# Autodesk Inventor assembly: Slides
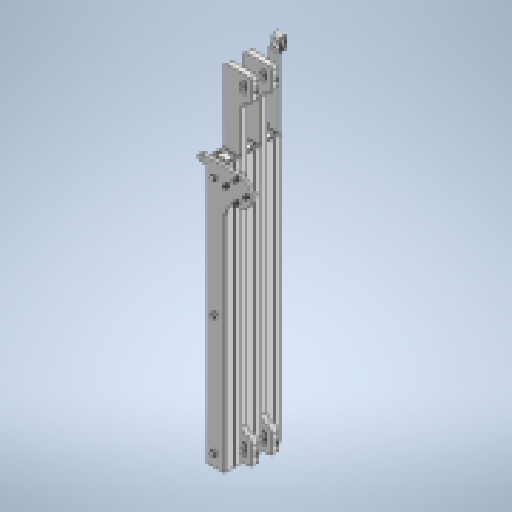
[picture p0: Inventor's stored thumbnail of the model, 512x512]
Saved by Autodesk Inventor 2023 (Build 270158000, 158)
## iProperties
Created: 2022-09-10
Part Number: Slides
Document SubType Name: Assembly
Designer: deli
Author: deli
## Documents named in this file (11)
- C:\Users\deli\OneDrive - Eastside Preparatory School\FTC\8103-power-play\CAD\Slides.iam
- C:\Users\deli\OneDrive - Eastside Preparatory School\FTC\8103-power-play\CAD\FTC-parts\Middle Slide.ipt
- C:\Users\deli\OneDrive - Eastside Preparatory School\FTC\8103-power-play\CAD\FTC-parts\KC-362-30.iam
- C:\Users\deli\OneDrive - Eastside Preparatory School\FTC\8103-power-play\CAD\FTC-parts\LBracket.ipt
- C:\Users\deli\OneDrive - Eastside Preparatory School\FTC\8103-power-play\CAD\ServoMountPlate.ipt
- C:\Users\deli\OneDrive - Eastside Preparatory School\FTC\8103-power-play\CAD\FTC-parts\goBILDA\m3LockNute.ipt
- C:\Users\deli\OneDrive - Eastside Preparatory School\FTC\8103-power-play\CAD\FTC-parts\goBILDA\2800-0004-0008.ipt
- C:\Users\deli\OneDrive - Eastside Preparatory School\FTC\8103-power-play\CAD\FTC-parts\M3\hex_socket_button_head_M3x20.ipt
- C:\Users\deli\OneDrive - Eastside Preparatory School\FTC\8103-power-play\CAD\FTC-parts\LongRobotics\3x12x4mm-bearing.ipt
- C:\Users\deli\OneDrive - Eastside Preparatory School\FTC\8103-power-play\CAD\FTC-parts\goBILDA\2812-0004-0007.ipt
- C:\Users\deli\OneDrive - Eastside Preparatory School\FTC\8103-power-play\CAD\FTC-parts\goBILDA\3408-0001-0001 assembly.ipt
## Components (27 placed, 10 different names)
1. Middle Slide:1
2. KC-362-30:1 [sub-assembly]
3. Middle Slide:2
4. KC-362-30:2 [sub-assembly]
5. KC-362-30:3 [sub-assembly] — Mate:15, Mate:16, Mate:17
6. LBracket:1 — Mate:18, Mate:19, Mate:20, Mate:21, Mate:52, Mate:53, Mate:54, Mate:55, Mate:56, Mate:57, Flush:2
7. ServoMountPlate:1 — Mate:15, Mate:16, Mate:17, Mate:22, Mate:23, Mate:24, Mate:25, Mate:26, Mate:27, Mate:28, Mate:29, Mate:46, Mate:47, Mate:48, Mate:49, Mate:50, Mate:51
8. m3LockNute:1 — Mate:18, Mate:19
9. m3LockNute:2 — Mate:20, Mate:21
10. 2800-0004-0008:1 — Mate:22, Mate:28
11. 2800-0004-0008:2 — Mate:24, Mate:27
12. 2800-0004-0008:3 — Mate:23, Mate:29
13. 2800-0004-0008:4 — Mate:25, Mate:26
14. hex_socket_button_head_M3x20:1
15. hex_socket_button_head_M3x20:2
16. hex_socket_button_head_M3x20:3
17. hex_socket_button_head_M3x20:4
18. 3x12x4mm-bearing:1
19. 3x12x4mm-bearing:2
20. 3x12x4mm-bearing:3
21. 3x12x4mm-bearing:4
22. m3LockNute:3 — Mate:46, Mate:47
23. m3LockNute:4 — Mate:48, Mate:51
24. m3LockNute:5 — Mate:49, Mate:50
25. 2812-0004-0007:1 — Mate:54, Mate:55
26. 2812-0004-0007:2 — Mate:52, Mate:53
27. 3408-0001-0001 assembly:1 — Mate:56, Mate:57, Flush:2
## Relationships (59: Mate 57, Flush 2)
- [Mate]: Middle Slide:1 ↔ KC-362-30:1
- [Mate]: Middle Slide:1 ↔ KC-362-30:1
- [Mate]: Middle Slide:1 ↔ KC-362-30:1
- [Mate]: Middle Slide:2 ↔ KC-362-30:2
- [Mate]: Middle Slide:2 ↔ KC-362-30:2
- [Mate]: Middle Slide:2 ↔ KC-362-30:2
- [Mate]: Middle Slide:1 ↔ KC-362-30:2
- [Mate]: Middle Slide:1 ↔ KC-362-30:2
- [Mate]: Middle Slide:1 ↔ KC-362-30:2
- [Mate]: Middle Slide:2 ↔ KC-362-30:3
- [Mate]: Middle Slide:2 ↔ KC-362-30:3
- [Mate]: Middle Slide:2 ↔ KC-362-30:3
- [Mate]: KC-362-30:1 ↔ LBracket:1
- [Flush]: KC-362-30:1 ↔ LBracket:1
- [Mate] (7 mm): KC-362-30:1 ↔ LBracket:1
- Mate:15: KC-362-30:3 ↔ ServoMountPlate:1
- Mate:16: KC-362-30:3 ↔ ServoMountPlate:1
- Mate:17: KC-362-30:3 ↔ ServoMountPlate:1
- Mate:18: LBracket:1 ↔ m3LockNute:1
- Mate:19: LBracket:1 ↔ m3LockNute:1
- Mate:20: LBracket:1 ↔ m3LockNute:2
- Mate:21: LBracket:1 ↔ m3LockNute:2
- Mate:22: ServoMountPlate:1 ↔ 2800-0004-0008:1
- Mate:23: ServoMountPlate:1 ↔ 2800-0004-0008:3
- Mate:24: ServoMountPlate:1 ↔ 2800-0004-0008:2
- Mate:25: ServoMountPlate:1 ↔ 2800-0004-0008:4
- Mate:26: ServoMountPlate:1 ↔ 2800-0004-0008:4
- Mate:27: ServoMountPlate:1 ↔ 2800-0004-0008:2
- Mate:28: ServoMountPlate:1 ↔ 2800-0004-0008:1
- Mate:29: ServoMountPlate:1 ↔ 2800-0004-0008:3
- [Mate]: Middle Slide:2 ↔ hex_socket_button_head_M3x20:3
- [Mate]: Middle Slide:1 ↔ hex_socket_button_head_M3x20:4
- [Mate]: Middle Slide:2 ↔ hex_socket_button_head_M3x20:2
- [Mate]: Middle Slide:1 ↔ hex_socket_button_head_M3x20:1
- [Mate]: Middle Slide:2 ↔ hex_socket_button_head_M3x20:3
- [Mate]: Middle Slide:1 ↔ hex_socket_button_head_M3x20:4
- [Mate]: Middle Slide:2 ↔ hex_socket_button_head_M3x20:2
- [Mate]: Middle Slide:1 ↔ hex_socket_button_head_M3x20:1
- [Mate]: hex_socket_button_head_M3x20:3 ↔ 3x12x4mm-bearing:1
- [Mate]: hex_socket_button_head_M3x20:4 ↔ 3x12x4mm-bearing:2
- [Mate] (1.175 mm): Middle Slide:2 ↔ 3x12x4mm-bearing:1
- [Mate] (1.175 mm): Middle Slide:1 ↔ 3x12x4mm-bearing:2
- [Mate] (1.175 mm): Middle Slide:1 ↔ 3x12x4mm-bearing:4
- [Mate]: hex_socket_button_head_M3x20:1 ↔ 3x12x4mm-bearing:4
- [Mate] (1.175 mm): Middle Slide:2 ↔ 3x12x4mm-bearing:3
- [Mate]: hex_socket_button_head_M3x20:2 ↔ 3x12x4mm-bearing:3
- Mate:46: ServoMountPlate:1 ↔ m3LockNute:3
- Mate:47: ServoMountPlate:1 ↔ m3LockNute:3
- Mate:48: ServoMountPlate:1 ↔ m3LockNute:4
- Mate:49: ServoMountPlate:1 ↔ m3LockNute:5
- Mate:50: ServoMountPlate:1 ↔ m3LockNute:5
- Mate:51: ServoMountPlate:1 ↔ m3LockNute:4
- Mate:52: LBracket:1 ↔ 2812-0004-0007:2
- Mate:53: LBracket:1 ↔ 2812-0004-0007:2
- Mate:54: LBracket:1 ↔ 2812-0004-0007:1
- Mate:55: LBracket:1 ↔ 2812-0004-0007:1
- Mate:56: LBracket:1 ↔ 3408-0001-0001 assembly:1
- Mate:57: LBracket:1 ↔ 3408-0001-0001 assembly:1
- Flush:2: LBracket:1 ↔ 3408-0001-0001 assembly:1
## Named parameters: d3_d0 = 0 mm, d4_d1 = 0 mm, d5_d2 = 0 mm
